# Autodesk Inventor assembly: Selection_Shaft Assy 4 Lanes
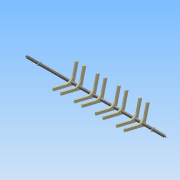
[picture p0: Inventor's stored thumbnail of the model, 180x180]
Saved by Autodesk Inventor 2018.1 (Build 221171000, 171)
## iProperties
Created: 2019-02-14
Part Number: Selection_Shaft Assy 4 Lanes
Document SubType Name: Assembly
Designer: James
Author: James
## Documents named in this file (4)
- C:\Users\admin\Desktop\Ball Sorting Machine\Ball-Sorting-Machine\Selection Sort\Selection - 4 Lanes\Selection_Shaft Assy 4 Lanes.iam
- C:\Users\admin\Desktop\Ball Sorting Machine\Ball-Sorting-Machine\Selection Sort\Selection_Shaft 1.ipt
- C:\Users\admin\Desktop\Ball Sorting Machine\Ball-Sorting-Machine\Selection Sort\Selection_Selector 1.ipt
- C:\Users\admin\Desktop\Ball Sorting Machine\Ball-Sorting-Machine\Timing Gate\BS 3673 - 6mm External Circlip.ipt
## Components (19 placed, 3 different names)
1. Selection_Shaft 1:1 — Flush:1, Flush:2, Flush:3, Mate:1, Mate:2, Flush:5, Flush:6, Mate:3, Mate:4, Mate:5, Mate:6, Mate:7, Mate:8, Mate:9, Mate:10
2. BS 3673 - 6mm External Circlip:11 — Mate:7, Mate:8, Flush:8
3. BS 3673 - 6mm External Circlip:12 — Mate:9, Mate:10, Flush:7, Flush:8
4. BS 3673 - 6mm External Circlip:2 — Mate:4, Mate:5, Flush:7, Flush:9
5. Selection_Selector 1:1 — Mate:2, Flush:4, Flush:5
6. BS 3673 - 6mm External Circlip:1 — Mate:3, Mate:6, Flush:9
7. Selection_Selector 1:2 — Mate:1, Flush:4, Flush:6
8. BS 3673 - 6mm External Circlip:3
9. Selection_Selector 1:3
10. BS 3673 - 6mm External Circlip:4
11. Selection_Selector 1:4
12. BS 3673 - 6mm External Circlip:5
13. Selection_Selector 1:5
14. BS 3673 - 6mm External Circlip:6
15. Selection_Selector 1:6
16. BS 3673 - 6mm External Circlip:7
17. Selection_Selector 1:7
18. BS 3673 - 6mm External Circlip:8
19. Selection_Selector 1:8
## Component patterns: (4 elements, first: BS 3673 - 6mm External Circlip:2 + Selection_Selector 1:1 + BS 3673 - 6mm External Circlip:1 + Selection_Selector 1:2)
## Relationships (19: Mate 10, Flush 9)
- Flush:1: Selection_Shaft 1:1
- Flush:2: Selection_Shaft 1:1
- Flush:3: Selection_Shaft 1:1
- Mate:1: Selection_Shaft 1:1 ↔ Selection_Selector 1:2
- Mate:2: Selection_Shaft 1:1 ↔ Selection_Selector 1:1
- Flush:4: Selection_Selector 1:1 ↔ Selection_Selector 1:2
- Flush:5: Selection_Shaft 1:1 ↔ Selection_Selector 1:1
- Flush:6: Selection_Shaft 1:1 ↔ Selection_Selector 1:2
- Mate:3: Selection_Shaft 1:1 ↔ BS 3673 - 6mm External Circlip:1
- Mate:4: Selection_Shaft 1:1 ↔ BS 3673 - 6mm External Circlip:2
- Mate:5: Selection_Shaft 1:1 ↔ BS 3673 - 6mm External Circlip:2
- Mate:6: Selection_Shaft 1:1 ↔ BS 3673 - 6mm External Circlip:1
- Mate:7: Selection_Shaft 1:1 ↔ BS 3673 - 6mm External Circlip:11
- Mate:8: Selection_Shaft 1:1 ↔ BS 3673 - 6mm External Circlip:11
- Mate:9: Selection_Shaft 1:1 ↔ BS 3673 - 6mm External Circlip:12
- Mate:10: Selection_Shaft 1:1 ↔ BS 3673 - 6mm External Circlip:12
- Flush:7: BS 3673 - 6mm External Circlip:12 ↔ BS 3673 - 6mm External Circlip:2
- Flush:8: BS 3673 - 6mm External Circlip:11 ↔ BS 3673 - 6mm External Circlip:12
- Flush:9: BS 3673 - 6mm External Circlip:2 ↔ BS 3673 - 6mm External Circlip:1
